# Autodesk Inventor assembly: ApparatusMasterAssemV5
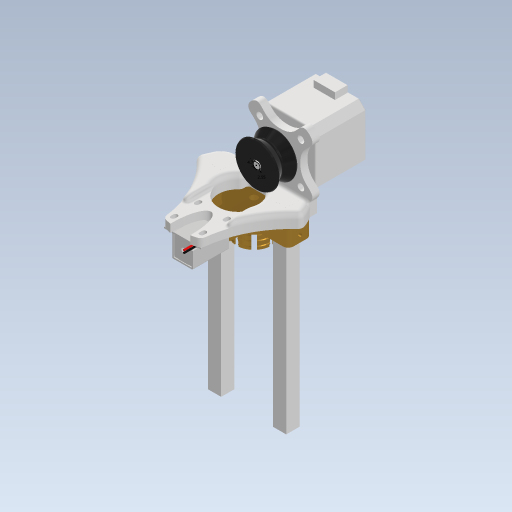
[picture p0: Inventor's stored thumbnail of the model, 512x512]
Saved by Autodesk Inventor 2023 (Build 270158000, 158)
## iProperties
Created: 2022-10-17
Part Number: ApparatusMasterAssemV5
Document SubType Name: Assembly
Designer: Dave
Author: Dave
## Documents named in this file (7)
- C:\Users\Dave\Documents\GrabCAD\Chalk Bot\Chalkbot1.0\Apparatus\V5\ApparatusMasterAssemV5.iam
- C:\Users\Dave\Documents\GrabCAD\Chalk Bot\Chalkbot1.0\Apparatus\V5\Slider V9 (4mm pitch).ipt
- C:\Users\Dave\Documents\GrabCAD\Chalk Bot\Chalkbot1.0\Apparatus\V5\Vertical Pole.ipt
- C:\Users\Dave\Documents\GrabCAD\Chalk Bot\Chalkbot1.0\Apparatus\V5\Solenoid Support.ipt
- C:\Users\Dave\Documents\GrabCAD\Chalk Bot\Chalkbot1.0\Apparatus\V5\Solenoid Lock.ipt
- C:\Users\Dave\Documents\GrabCAD\Chalk Bot\Chalkbot1.0\Apparatus\V5\Motor Model.ipt
- C:\Users\Dave\Documents\GrabCAD\Chalk Bot\Chalkbot1.0\Apparatus\V3\Stepper Attachments\Stepper Pulley V12.ipt
## Components (7 placed, 6 different names)
1. Slider V8 (4mm pitch):1 — Mate:8, Mate:9
2. Vertical Pole:1 — Mate:9, Angle:1
3. Vertical Pole:2 — Mate:8
4. Solenoid Support:1 — Mate:13, Mate:14, Mate:15, Insert:1
5. Solenoid Lock:1 — Mate:13, Mate:14, Mate:15
6. Motor Model:1 — Insert:1, Angle:1, Mate:16, Flush:1
7. Stepper Pulley V12:1 — Mate:16, Flush:1
## Relationships (9: Mate 6, Insert 1, Angle 1, Flush 1)
- Mate:8 (0.25 mm): Slider V8 (4mm pitch):1 ↔ Vertical Pole:2
- Mate:9 (0.25 mm): Slider V8 (4mm pitch):1 ↔ Vertical Pole:1
- Mate:13: Solenoid Support:1 ↔ Solenoid Lock:1
- Mate:14: Solenoid Support:1 ↔ Solenoid Lock:1
- Mate:15: Solenoid Support:1 ↔ Solenoid Lock:1
- Insert:1: Solenoid Support:1 ↔ Motor Model:1
- Angle:1 (0 deg): Vertical Pole:1 ↔ Motor Model:1
- Mate:16: Motor Model:1 ↔ Stepper Pulley V12:1
- Flush:1: Motor Model:1 ↔ Stepper Pulley V12:1
